# Autodesk Inventor assembly: Eslabon2
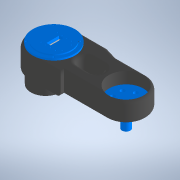
[picture p0: Inventor's stored thumbnail of the model, 180x180]
Saved by Autodesk Inventor 2021 (Build 250183000, 183)
## iProperties
Created: 2022-04-22
Part Number: Eslabon2
Document SubType Name: Assembly
Designer: Alcatraz
Author: Alcatraz
## Documents named in this file (7)
- F:\Tesis\TESIS\Matlab\Pruebas\Prueba3_Simulacion2\Eslabon2.iam
- F:\Tesis\TESIS\Eslabon_intermedio5_Parametrizado.ipt
- F:\Tesis\TESIS\Brida_5_parametrizado.ipt
- F:\Tesis\TESIS\Eje_3_parametrizado.ipt
- F:\Tesis\TESIS\rodamiento_dummie.ipt
- F:\Tesis\TESIS\AX-12A,18A,12W,MX-12W(stp)\AX-12A.iam
- F:\Tesis\TESIS\Tapa_eslabon.ipt
## Components (7 placed, 6 different names)
1. Eslabon_intermedio5_Parametrizado:1 — Coincidencia:4, Coincidencia:5, Coincidencia:6, Coincidencia:12, Coincidencia:13, Coincidencia:14, Coincidencia:15
2. Brida_5_parametrizado:1 — Coincidencia:9, Coincidencia:10, Coincidencia:11, Coincidencia:16
3. Eje_3_parametrizado:1 — Coincidencia:12, Coincidencia:13, Coincidencia:14
4. rodamiento_dummie:1 — Coincidencia:7, Coincidencia:8, Coincidencia:15, Coincidencia:16
5. rodamiento_dummie:2 — Coincidencia:7, Coincidencia:8
6. AX-12A:1 [sub-assembly] — Coincidencia:1, Coincidencia:2, Coincidencia:3, Coincidencia:9, Coincidencia:10, Coincidencia:11
7. Tapa_eslabon:1 — Coincidencia:1, Coincidencia:2, Coincidencia:3, Coincidencia:4, Coincidencia:5, Coincidencia:6
## Relationships (16: Mate 16)
- Coincidencia:1 [Mate]: AX-12A:1 ↔ Tapa_eslabon:1
- Coincidencia:2 [Mate]: AX-12A:1 ↔ Tapa_eslabon:1
- Coincidencia:3 [Mate]: AX-12A:1 ↔ Tapa_eslabon:1
- Coincidencia:4 [Mate]: Eslabon_intermedio5_Parametrizado:1 ↔ Tapa_eslabon:1
- Coincidencia:5 [Mate]: Eslabon_intermedio5_Parametrizado:1 ↔ Tapa_eslabon:1
- Coincidencia:6 [Mate]: Eslabon_intermedio5_Parametrizado:1 ↔ Tapa_eslabon:1
- Coincidencia:7 [Mate]: rodamiento_dummie:1 ↔ rodamiento_dummie:2
- Coincidencia:8 [Mate]: rodamiento_dummie:1 ↔ rodamiento_dummie:2
- Coincidencia:9 [Mate]: Brida_5_parametrizado:1 ↔ AX-12A:1
- Coincidencia:10 [Mate]: Brida_5_parametrizado:1 ↔ AX-12A:1
- Coincidencia:11 [Mate]: Brida_5_parametrizado:1 ↔ AX-12A:1
- Coincidencia:12 [Mate]: Eslabon_intermedio5_Parametrizado:1 ↔ Eje_3_parametrizado:1
- Coincidencia:13 [Mate]: Eslabon_intermedio5_Parametrizado:1 ↔ Eje_3_parametrizado:1
- Coincidencia:14 [Mate]: Eslabon_intermedio5_Parametrizado:1 ↔ Eje_3_parametrizado:1
- Coincidencia:15 [Mate]: Eslabon_intermedio5_Parametrizado:1 ↔ rodamiento_dummie:1
- Coincidencia:16 [Mate]: Brida_5_parametrizado:1 ↔ rodamiento_dummie:1
